# Autodesk Inventor assembly: main
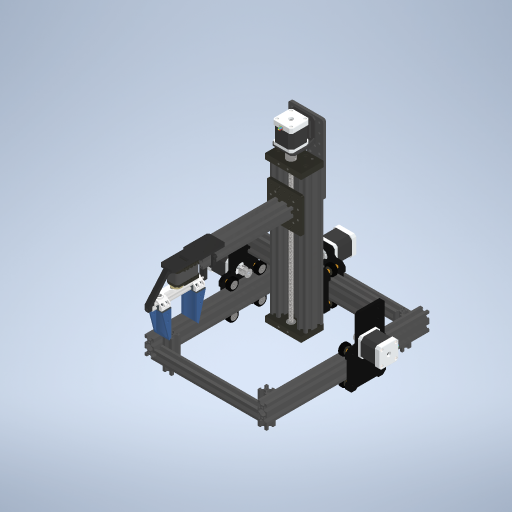
[picture p0: Inventor's stored thumbnail of the model, 512x512]
Saved by Autodesk Inventor 2024.2 (Build 282272000, 272)
## iProperties
Created: 2024-08-26
Part Number: main
Document SubType Name: Assembly
Designer: Admin
Author: 1:5
Title: Ensamble general
## Documents named in this file (6)
- C:\Users\Admin\Documents\GitHub\ManipuladorCartesiano\DiseñoMecánico\Assemblies\main_2.iam
- C:\Users\Admin\Documents\GitHub\ManipuladorCartesiano\DiseñoMecánico\Assemblies\AxisX.iam
- C:\Users\Admin\Documents\GitHub\ManipuladorCartesiano\DiseñoMecánico\Assemblies\AxisY.iam
- C:\Users\Admin\Documents\GitHub\ManipuladorCartesiano\DiseñoMecánico\Assemblies\AxisZ.iam
- C:\Users\Admin\Documents\GitHub\ManipuladorCartesiano\DiseñoMecánico\Assemblies\MovingPlate.iam
- C:\Users\Admin\Documents\GitHub\ManipuladorCartesiano\DiseñoMecánico\Assemblies\Claw.iam
## Components (5 placed, 5 different names)
1. AxisX:1 [sub-assembly] — Tangent:1, Tangent:2, Tangent:3
2. AxisY:1 [sub-assembly] — Tangent:1, Tangent:2, Tangent:3, Tangent:4, Tangent:5, Tangent:6, Tangent:7
3. AxisZ:1 [sub-assembly] — Tangent:4, Tangent:5, Tangent:6, Tangent:7, Mate:2, Flush:1
4. MovingPlate:1 [sub-assembly] — Mate:2, Flush:1, Mate:3, Flush:2, Mate:4
5. Claw:1 [sub-assembly] — Mate:3, Flush:2, Mate:4
## Relationships (12: Tangent 7, Mate 3, Flush 2)
- Tangent:1: AxisX:1 ↔ AxisY:1
- Tangent:2: AxisX:1 ↔ AxisY:1
- Tangent:3: AxisX:1 ↔ AxisY:1
- Tangent:4: AxisY:1 ↔ AxisZ:1
- Tangent:5: AxisY:1 ↔ AxisZ:1
- Tangent:6: AxisY:1 ↔ AxisZ:1
- Tangent:7: AxisY:1 ↔ AxisZ:1
- Mate:2: AxisZ:1 ↔ MovingPlate:1
- Flush:1 (1.425 mm): AxisZ:1 ↔ MovingPlate:1
- Mate:3: MovingPlate:1 ↔ Claw:1
- Flush:2: MovingPlate:1 ↔ Claw:1
- Mate:4 (1.6 mm): MovingPlate:1 ↔ Claw:1
